# Autodesk Inventor assembly: 041
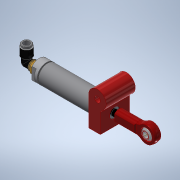
[picture p0: Inventor's stored thumbnail of the model, 180x180]
Saved by Autodesk Inventor 2020 (Build 240168000, 168)
## iProperties
Part Number: 041
Catalog Web Link: www.cadenas.de
Description: Original Line Standard Air Cylinders-Standard Air Cylinders
Vendor: BIMBA
Document SubType Name: Assembly
Designer: partserver
Manufacturer: BIMBA
Mass: 18.0554 g
Surface Area: 157.339 cm^2
Volume: 18.0554 cm^3
Density: 1 g/cm^3
Category: PARTsolutions
Company: BIMBA
PSOL_IDENT_0: {$CADENAS_DATA\23d-libs\bimba\bimba_brand\bimba_imperial\bimba_full_line\original_line_cylinders\sta
PSOL_IDENT_1: ndard_air_cylinders\standard_air_cylinder_asmtab.prj},314 {VTYP=3D},{STYP=ASSTAB},{NB=041},{LINA=041
PSOL_IDENT_2: },{NN=Original Line Standard Air Cylinders},{DATE=19.01.2022 10:19:38},{GEOMDATE=11.11.2021 07:31:43
PSOL_IDENT_3: },{VERSION=},{LINEID=50},{WBVAR=STROKE,ACTING,MNT,DER,NR,BM,CO,OO,VO,M,EE,EEL,K,Q,Y,G,T,HL,B,H,SER,S
PSOL_IDENT_4: R,NT,W,STPT1,STPT2,STPT3,STPT4,MB,PB,PRC,TB,MN},{WBNUMERIC=STROKE,EEL}  {NB=041},{LINA=041},{KT=DUMM
PSOL_IDENT_5: Y},{PN=041},{PNC=041},{PNA=(NO ACCESSORIES)},{PNAHELP=},{DASH=},{BORE1=0.75000000},{BORE=3/4\" (04)}
PSOL_IDENT_6: ,{BOREPN=04},{STROKE=1.000},{STROKEALG=[0.011:50/0.001]},{STROKE1=1.000},{ACTING=},{ACTINGALG= '' , '
PSOL_IDENT_7: Single Acting' , 'R' , 'Reverse Single Acting (R)' , 'D' , 'Double Acting (D)' },{ACTINGPN=},{MNT=},
PSOL_IDENT_8: {MNTALG= '' , 'Front Nose Mounting' , 'P' , 'Rear Pivot Mounting (P)' , 'BF' , 'Front Block Mounting
PSOL_IDENT_9: (BF)' , 'BR' , 'Rear Block Mounting for Vertical Positioning (BR)' , 'BFT' , 'Front Block Trunnion
PSOL_IDENT_10: Mounting (BFT)' , 'BRT' , 'Rear Block Trunnion Mounting (BRT)' , 'A' , 'Double End Mounting with Bra
PSOL_IDENT_11: ckets and Adjustable Stroke (A)' , 'AP' , 'Rear Pivot Mounting with Adjustable Stroke (AP)' },{TYPE=
PSOL_IDENT_12: },{MNTPN=},{DER=},{DERALG= '' , 'N/A' },{NR=},{NRALG= '' , 'Round (Standard)' , 'NR' , 'Non-rotating
PSOL_IDENT_13: - Hexagon Rod' },{NRPN=},{BM=},{BMALG= '' , 'Without Built-in Midget 3-Way Solenoid Operated Valve'
PSOL_IDENT_14: , 'LS' , 'With LS Series Solenoid Valve [LS]' },{BMPN=},{CO=},{COALG= '' , 'N/A' },{OO=},{OOALG= ''
PSOL_IDENT_15: , 'N/A' },{OOPN=},{VO=Z},{VOALG= 'Z' , 'N/A' },{VOPN=},{OOVOPN=},{M=},{MALG= '', 'Without Magnet', '
PSOL_IDENT_16: M', 'With Magnet' },{EE=},{EEL=0.000},{EEMAX=49.0000},{EEALG= '', 'Without Extra Extension', 'EE', '
PSOL_IDENT_17: With Extra Extension' },{EELALG=0},{EEPN=},{EEPN1=0.000},{K=},{KALG= '' , 'N/A' },{KPN=},{Q=},{QALG=
PSOL_IDENT_18: '' , 'Standard Port' , 'Q' , 'Side Port' },{QPN=},{Y=},{YALG= '' , 'N/A' },{YPN=},{YCON=},{F=},{FAL
PSOL_IDENT_19: G= '', 'Non-Coated (Standard)', 'F', 'Molycoated' },{FPN=},{G=},{GPN=},{GPN99=},{T=},{TALG= '' , 'St
PSOL_IDENT_20: andard -20° to 200°F (-29° to 95°C)' , 'N' , 'Low Temperature' , 'V' , 'High Temperature' },{NPN=},{
PSOL_IDENT_21: VPN=},{HL=},{HLALG= '' , 'N/A' },{B=},{BALG= '', 'W/out Bumpers' , 'B' , 'W/ Bumpers' },{BPN=},{H=},
PSOL_IDENT_22: {HALG= '', 'W/ Standard Spring (Relaxed 3 lbs./Compressed 6 lbs.)', 'H', 'W/ Heavy Spring (Relaxed 4
PSOL_IDENT_23: lbs./Compressed 10 lbs.)' },{HPN=},{SER=},{SERALG= '' , 'N/A' },{SR=C},{SRALG= 'C' , 'Standard Blac
PSOL_IDENT_24: kened Carbon Steel' , 'SR' , 'Stainless Steel [SR]' },{SRPN=},{SRCON=1},{NT=},{NTPN=},{W=},{WALG= ''
PSOL_IDENT_25: , 'N/A' },{WPN=},{E=},{EALG= '' , 'Standard Seals/Lube' , 'E' , 'Non-Lube Seals/Lube' },{EPN=},{ST=
PSOL_IDENT_26: },{STALG= '' , 'N/A' },{STPT1=},{STPT1ALG= '' , 'N/A' },{STPT2=},{STPT2ALG= '' , 'N/A' },{STPT3=},{S
PSOL_IDENT_27: TPT3ALG= '' , 'N/A' },{STPT4=},{STPT4ALG= '' , 'N/A' },{STPN=},{MB=},{MBALG= '' , 'Without Mounting
PSOL_IDENT_28: Bracket' , 'F,D-226' , 'D-226 (front)' },{MBPN=},{MBPNALL=D-226},{MBPNALLREAR=},{PB=},{PBALG= '' , '
PSOL_IDENT_29: N/A' },{PBPN=},{PBPNALL=},{PRC=},{PRCALG= '' , 'W/out Pivot Rod Clevis' , 'F,D-166-3' , 'D-166-3 (fr
PSOL_IDENT_30: ont)' },{PRCPN=},{PRCPNALL=D-166-3},{TB=},{TBALG= '' , 'N/A' },{TBPN=},{TBPNALL=},{MN=},{MNALG= '' ,
PSOL_IDENT_31: 'N/A' },{MNPN=},{MNCONF=},{MNCONR=},{TLEN=2.2560},{FRAC=3.8800},{RGCON=},{RGDACCON=},{RHCON=},{RHCO
PSOL_IDENT_32: N1=},{RHCONON=1},{RHACCON=},{FNUTCON=1},{RNUTCON=0},{FNUTPN=D-98},{RNUTPN=},{FNUTTRANS=0.0000},{RNUT
PSOL_IDENT_33: TRANS=0.0000},{VHOLECON=2},{A1=0.8750},{A1N=0.8750},{A1P=1.5940},{A1B=1.5940},{A4=0.3130},{A4N=0.313
PSOL_IDENT_34: 0},{A4P=0.2525},{A5=0.0300},{A1H=0.531},{A1NH=0.5310},{A1PH=1.5940},{A1BH=1.0940},{A1SH=1.2190},{A2H=
PSOL_IDENT_35: 0.2190},{A2NH=0.2190},{LENGTH=1.5000},{LENGTH1=1.5000},{LENGTH2=3.0300},{MUL=1.6900},{MUL11=1.6900},
PSOL_IDENT_36: {MUL22=2.69},{MUL33=1.6900},{MUL2=1.6900},{MUL211=1.6900},{MUL222=2.6900},{MUL233=1.6900},{SSS=2.000
PSOL_IDENT_37: 0},{RGLEN=0.5920},{RHLEN=0.3420},{SSS1=2.0000},{A13=1.3120},{DIF=0.0000},{G5=0.6250},{ON=0},{SSADD=0
PSOL_IDENT_38: .0000},{BADD=0.0000},{MADD=0.0000},{NVADD=0.0000},{TRACKL=1.9660},{TRACKCON=D-74168},{TRIMCON=0},{TR
PSOL_IDENT_39: IMCON1=0},{PINCON=},{FSPACE=0.5571},{SPACE=0.0536},{TEXT=0.0938},{S1=1.0000},{D1=0.8050},{D1N=0.8050
PSOL_IDENT_40: },{D1B=0.8625},{D1P=0.8325},{FA=0.750},{RA=0.0000},{PPATH=standard_air_cylinder_asmtpl.prj},{MATALGH
PSOL_IDENT_41: TML=<b>Standard Original Line:</b><dl><dt>Rod:</dt><dd>- Stainless Steel</dd><dd>&nbsp;&nbsp;(5/16 9
PSOL_IDENT_42: /16 Bores)</dd><dd>- High Strength Carbon Steel</dd><dd>&nbsp;&nbsp;(3/4 3 Bore)</dd><dd>- Stainless
PSOL_IDENT_43: Steel</dd><dd>&nbsp;&nbsp;(X style DXP/DX/DXDE)</dd><dt>Bearings:</dt><dd>- Sintered Bronze</dd><dt
PSOL_IDENT_44: >Body:</dt><dd>- 304 Stainless Steel</dd><dt>End Caps:</dt><dd>- Aluminum</dd><dt>Seals:</dt><dd>- B
PSOL_IDENT_45: una N</dd></dl>},{ASSCFGPRA=04},{MBPNA=},{MNPNA=},{PRCPNA=},{ASSOPTACC=STPT4},{A=3.19},{HADD=0.0000}
PSOL_IDENT_46: ,{WFL=0.25},{QADD=0.000},{QADD1=0.440},{TEST=1.0000},{MNTB=},{STDNUTF=1},{STDNUTR=0},{STRK2D=0},{X2D=
PSOL_IDENT_47: 2},{STROKESW=1.000},{EESW=0.000},{FCD=0},{BCD=0},{RCD=0},{CUSTADD=0.000},{FT=1/4-28 UNF-2A},{FT1=1/4
PSOL_IDENT_48: -28 UNF-2A},{FT2=5/8-18 UNF-2A},{PORT=1/8 NPT},{FT11=1/2-20 UNF-2A},{FT12=5/8-18 UNF-2A},{B1=}
NB: 041
NN: Original Line Standard Air Cylinders
NT: Threaded (Standard)
NBSYN: $PNC.
LINA: 041
CATALOG: Bimba Products
PN: 041
PNA: (NO ACCESSORIES)
BORE: 3/4" (04)
STROKE: 1
ACTING: Single [Standard]
MNT: Front Nose
DER: N/A
NR: Round (Standard)
BM: Without Built-in Midget 3-Way Solenoid Operated Valve
CO: N/A
OO: N/A
VO: N/A
M: Without Magnet
EE: Without Extra Extension
EEL: 0
K: N/A
Q: Standard Port
Y: N/A
G: Standard Lube
T: Standard -20° to 200°F (-29° to 95°C)
HL: N/A
B: W/out Bumpers
H: W/ Standard Spring (Relaxed 3 lbs./Compressed 6 lbs.)
SER: N/A
SR: Standard Blackened Carbon Steel
W: N/A
STPT1: N/A
STPT2: N/A
STPT3: N/A
STPT4: N/A
MB: Without Mounting Bracket
PB: N/A
PRC: W/out Pivot Rod Clevis
TB: N/A
MN: N/A
A: 3.19
SUPPLIER: BIMBA
ARTICLENO: 041
BOMINFO: 041
CREATOR: CADENAS GmbH
Title: 041
Author: Cadenas PARTsolutions
Comments: Standard Air Cylinders
## Documents named in this file (9)
- T:\EIT\2022 Rapid React\COMMON PARTS\AIR CYLINDERS\BIMBA_041\AIS2020\041.iam
- T:\EIT\2022 Rapid React\COMMON PARTS\AIR CYLINDERS\BIMBA_041\AIS2020\041C0000000_0_dummy.ipt
- T:\EIT\2022 Rapid React\COMMON PARTS\AIR CYLINDERS\BIMBA_041\AIS2020\04000-0_rod_guide.ipt
- T:\EIT\2022 Rapid React\COMMON PARTS\AIR CYLINDERS\BIMBA_041\AIS2020\04-2_2562C.ipt
- T:\EIT\2022 Rapid React\COMMON PARTS\AIR CYLINDERS\BIMBA_041\AIS2020\040000_rear_head.ipt
- T:\EIT\2022 Rapid React\COMMON PARTS\AIR CYLINDERS\BIMBA_041\AIS2020\C-0410000_rod.ipt
- T:\EIT\2022 Rapid React\COMMON PARTS\AIR CYLINDERS\TieRod End\60685K321_PTFE-LINED ALUMINUM BALL JOINT ROD END.ipt
- T:\EIT\2022 Rapid React\SHOOTER\SH-ACM-001.ipt
- T:\EIT\2022 Rapid React\COMMON PARTS\AIR CYLINDERS\5779K151_PUSH-TO-CONNECT TUBE FITTING FOR AIR.ipt
## Components (8 placed, 8 different names)
1. 041C0000000_0_dummy:1
2. 04000-0_rod_guide:1 — Insert:1, Insert:3
3. 04-2_2562C:1
4. 040000_rear_head:1 — Angle:1, Insert:4
5. C-0410000_rod:1 — Insert:1, Insert:2
6. 60685K321_PTFE-LINED ALUMINUM BALL JOINT ROD END:1 — Insert:2, Angle:1, Angle:2
7. SH-ACM-001:1 — Insert:3, Angle:2
8. 5779K151_PUSH-TO-CONNECT TUBE FITTING FOR AIR:1 — Insert:4
## Relationships (6: Insert 4, Angle 2)
- Insert:1: 04000-0_rod_guide:1 ↔ C-0410000_rod:1
- Insert:2 (5 mm): C-0410000_rod:1 ↔ 60685K321_PTFE-LINED ALUMINUM BALL JOINT ROD END:1
- Angle:1 (0 deg): 040000_rear_head:1 ↔ 60685K321_PTFE-LINED ALUMINUM BALL JOINT ROD END:1
- Insert:3: 04000-0_rod_guide:1 ↔ SH-ACM-001:1
- Angle:2 (0 deg): 60685K321_PTFE-LINED ALUMINUM BALL JOINT ROD END:1 ↔ SH-ACM-001:1
- Insert:4 (2 mm): 040000_rear_head:1 ↔ 5779K151_PUSH-TO-CONNECT TUBE FITTING FOR AIR:1
